# Autodesk Inventor assembly: 1 cell
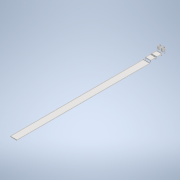
[picture p0: Inventor's stored thumbnail of the model, 180x180]
Saved by Autodesk Inventor 2020 (Build 240168000, 168)
## iProperties
Created: 2019-09-26
Part Number: 1 cell
Document SubType Name: Assembly
Designer: Abbas
Author: Abbas
## Documents named in this file (6)
- D:\Projects\aquaponic\Inventor\1 cell.iam
- D:\Projects\aquaponic\Inventor\fish tank 1.ipt
- D:\Projects\aquaponic\Inventor\swirl filter.ipt
- D:\Projects\aquaponic\Inventor\mineralisation.ipt
- D:\Projects\aquaponic\Inventor\grow bed.ipt
- D:\Projects\aquaponic\Inventor\dwc.ipt
## Components (6 placed, 5 different names)
1. fish tank 1:1
2. swirl filter:1 — Angle:1
3. mineralisation:1 — Angle:1
4. grow bed:1
5. grow bed:2
6. dwc:1
## Relationships (1: Angle 1)
- Angle:1 (0 deg): swirl filter:1 ↔ mineralisation:1
